# Autodesk Inventor assembly: immersion_chamber
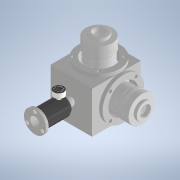
[picture p0: Inventor's stored thumbnail of the model, 180x180]
Saved by Autodesk Inventor 2021 (Build 250183000, 183)
## iProperties
Created: 2021-06-16
Part Number: immersion_chamber
Document SubType Name: Assembly
Designer: MicroscopyInnovation
Author: MicroscopyInnovation
## Documents named in this file (6)
- C:\Users\MicroscopyInnovation\Documents\Inventor\NatProtocolsManuscript\immersion_chamber_assembly.iam
- C:\Users\MicroscopyInnovation\Documents\Inventor\NatProtocolsManuscript\immersion_chamber_bath.ipt
- C:\Users\MicroscopyInnovation\Documents\Inventor\NatProtocolsManuscript\immersion_chamber_plate.ipt
- C:\Users\MicroscopyInnovation\Documents\Inventor\NatProtocolsManuscript\general_TR1.ipt
- C:\Users\MicroscopyInnovation\Documents\Inventor\NatProtocolsManuscript\general_PH1.5E.ipt
- C:\Users\MicroscopyInnovation\Documents\Inventor\NatProtocolsManuscript\54_10_12_multi_immersion_objective.ipt
## Components (7 placed, 5 different names)
1. immersion_chamber_bath:1 — Mate:1, Mate:2, Mate:3, Mate:4, Mate:5, Mate:6, Mate:7, Mate:8, Mate:9, Mate:11, Mate:12, Mate:13
2. immersion_chamber_plate:1 — Mate:1, Mate:2, Mate:3, Mate:4
3. immersion_chamber_plate:2 — Mate:5, Mate:6, Mate:7
4. general_TR1:1 — Mate:8, Mate:9, Mate:10
5. general_PH1.5E:1 — Mate:10, Mate:11
6. 54_10_12_multi_immersion_objective:1 — Mate:12, Mate:14, Mate:15
7. 54_10_12_multi_immersion_objective:2 — Mate:13, Mate:14, Mate:15
## Relationships (15: Mate 15)
- Mate:1: immersion_chamber_bath:1 ↔ immersion_chamber_plate:1
- Mate:2: immersion_chamber_bath:1 ↔ immersion_chamber_plate:1
- Mate:3: immersion_chamber_bath:1 ↔ immersion_chamber_plate:1
- Mate:4: immersion_chamber_bath:1 ↔ immersion_chamber_plate:1
- Mate:5: immersion_chamber_bath:1 ↔ immersion_chamber_plate:2
- Mate:6: immersion_chamber_bath:1 ↔ immersion_chamber_plate:2
- Mate:7: immersion_chamber_bath:1 ↔ immersion_chamber_plate:2
- Mate:8: immersion_chamber_bath:1 ↔ general_TR1:1
- Mate:9: immersion_chamber_bath:1 ↔ general_TR1:1
- Mate:10: general_TR1:1 ↔ general_PH1.5E:1
- Mate:11 (10 mm): immersion_chamber_bath:1 ↔ general_PH1.5E:1
- Mate:12: immersion_chamber_bath:1 ↔ 54_10_12_multi_immersion_objective:1
- Mate:13: immersion_chamber_bath:1 ↔ 54_10_12_multi_immersion_objective:2
- Mate:14: 54_10_12_multi_immersion_objective:1 ↔ 54_10_12_multi_immersion_objective:2
- Mate:15: 54_10_12_multi_immersion_objective:1 ↔ 54_10_12_multi_immersion_objective:2
